# Autodesk Inventor assembly: triangle_brace_mirrored
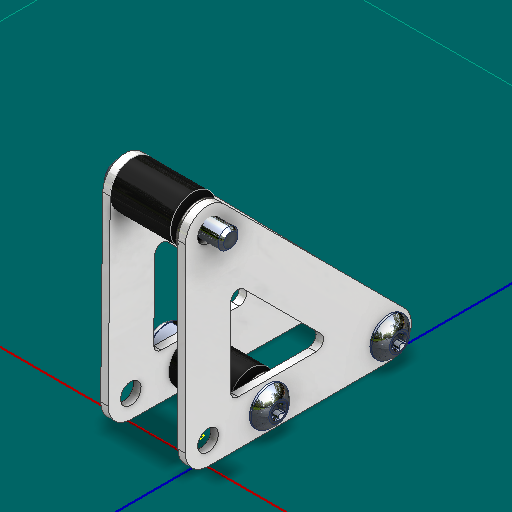
[picture p0: Inventor's stored thumbnail of the model, 512x512]
Saved by Autodesk Inventor 2025 (Build 290162000, 162)
## iProperties
Created: 2024-08-19
Part Number: triangle_brace_mirrored
Document SubType Name: Assembly
Designer: averey
Author: averey
## Documents named in this file (9)
- C:\Users\avere\vex_robotics_high_stakes\hardware\cad\ATLAS\tower\structure\triangle_brace_mirrored.iam
- C:\Users\avere\vex_robotics_high_stakes\hardware\cad\ATLAS\chassis\structure\custom_parts\right_angle_gusset.ipt
- C:\Users\avere\vex_robotics_high_stakes\hardware\cad\VEX-CAD-Inventor\Motion\Spacers\Spacer Nylon .375 OD\NSpacer .375 OD x .500.ipt
- C:\Users\avere\vex_robotics_high_stakes\hardware\cad\VEX-CAD-Inventor\Motion\Spacers\Spacer Nylon .375 OD.ipt
- C:\Users\avere\vex_robotics_high_stakes\hardware\cad\VEX-CAD-Inventor\Motion\Spacers\Washer Steel\SWasher .375 OD x .015625.ipt
- C:\Users\avere\vex_robotics_high_stakes\hardware\cad\VEX-CAD-Inventor\Motion\Spacers\Washer Steel.ipt
- C:\Users\avere\vex_robotics_high_stakes\hardware\cad\VEX-CAD-Inventor\Structure\Hardware\Screw Steel - Star\SScrew Star Smooth .875.ipt
- C:\Users\avere\vex_robotics_high_stakes\hardware\cad\VEX-CAD-Inventor\Structure\Hardware\Screw Steel - Star.ipt
- C:\Users\avere\vex_robotics_high_stakes\hardware\cad\VEX-CAD-Inventor\Structure\Hardware\Nut Thin Nylock.ipt
## Components (13 placed, 5 different names)
1. right_angle_gusset:1 — Insert:15, Insert:17, Insert:19, Insert:20, Insert:24, Insert:26
2. right_angle_gusset:2 — Mate:2, Insert:14, Insert:16, Insert:18, Insert:21, Insert:25
3. NSpacer .375 OD x .500:1 — Insert:19
4. NSpacer .375 OD x .500:2 — Insert:17
5. NSpacer .375 OD x .500:3 — Insert:24
6. SWasher .375 OD x .015625:1 — Insert:18
7. SWasher .375 OD x .015625:2 — Insert:25
8. SWasher .375 OD x .015625:3 — Insert:16
9. SScrew Star Smooth .875:1 — Insert:26
10. SScrew Star Smooth .875:2 — Insert:21
11. SScrew Star Smooth .875:3 — Insert:14
12. Nut Thin Nylock:1 — Insert:20
13. Nut Thin Nylock:2 — Insert:15
## Relationships (13: Insert 12, Mate 1)
- [Insert] (14.6844 mm): right_angle_gusset:1 ↔ right_angle_gusset:2
- Mate:2: right_angle_gusset:2
- Insert:14: right_angle_gusset:2 ↔ SScrew Star Smooth .875:3
- Insert:15: right_angle_gusset:1 ↔ Nut Thin Nylock:2
- Insert:16: right_angle_gusset:2 ↔ SWasher .375 OD x .015625:3
- Insert:17: right_angle_gusset:1 ↔ NSpacer .375 OD x .500:2
- Insert:18: right_angle_gusset:2 ↔ SWasher .375 OD x .015625:1
- Insert:19: right_angle_gusset:1 ↔ NSpacer .375 OD x .500:1
- Insert:20: right_angle_gusset:1 ↔ Nut Thin Nylock:1
- Insert:21: right_angle_gusset:2 ↔ SScrew Star Smooth .875:2
- Insert:24: right_angle_gusset:1 ↔ NSpacer .375 OD x .500:3
- Insert:25: right_angle_gusset:2 ↔ SWasher .375 OD x .015625:2
- Insert:26: right_angle_gusset:1 ↔ SScrew Star Smooth .875:1
